# Autodesk Inventor assembly: Colmeia
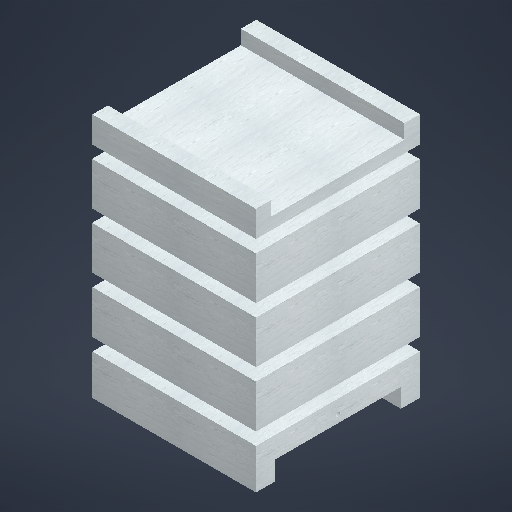
[picture p0: Inventor's stored thumbnail of the model, 512x512]
Saved by Autodesk Inventor 2027 (Build 310192000, 192)
## iProperties
Created: 2026-10-01
Part Number: Colmeia
Document SubType Name: Assembly
Designer: EspacoMaker
Author: EspacoMaker
## Documents named in this file (5)
- C:\Users\EspacoMaker\Documents\PeterIgnatious\BeeBox\3dFiles\Colmeia.iam
- C:\Users\EspacoMaker\Documents\PeterIgnatious\BeeBox\3dFiles\FundoColmeia.ipt
- C:\Users\EspacoMaker\Documents\PeterIgnatious\BeeBox\3dFiles\NinhoColmeia.ipt
- C:\Users\EspacoMaker\Documents\PeterIgnatious\BeeBox\3dFiles\Melgueira-Sobreninho.ipt
- C:\Users\EspacoMaker\Documents\PeterIgnatious\BeeBox\3dFiles\Tampa.ipt
## Components (5 placed, 4 different names)
1. FundoColmeia:1 — Coincidente:1, Alinhado:1, Alinhado:2
2. NinhoColmeia:1 — Coincidente:1, Alinhado:1, Alinhado:2, Coincidente:2, Alinhado:3, Alinhado:4
3. Melgueira-Sobreninho:1 — Coincidente:2, Alinhado:3, Alinhado:4, Coincidente:3, Alinhado:5, Alinhado:6
4. Melgueira-Sobreninho:2 — Coincidente:3, Alinhado:5, Alinhado:6, Coincidente:4, Alinhado:7, Alinhado:8
5. Tampa:1 — Coincidente:4, Alinhado:7, Alinhado:8
## Relationships (12: Flush 8, Mate 4)
- Coincidente:1 [Mate] (20 mm): FundoColmeia:1 ↔ NinhoColmeia:1
- Alinhado:1 [Flush]: FundoColmeia:1 ↔ NinhoColmeia:1
- Alinhado:2 [Flush]: FundoColmeia:1 ↔ NinhoColmeia:1
- Coincidente:2 [Mate] (20 mm): NinhoColmeia:1 ↔ Melgueira-Sobreninho:1
- Alinhado:3 [Flush]: NinhoColmeia:1 ↔ Melgueira-Sobreninho:1
- Alinhado:4 [Flush]: NinhoColmeia:1 ↔ Melgueira-Sobreninho:1
- Coincidente:3 [Mate] (20 mm): Melgueira-Sobreninho:1 ↔ Melgueira-Sobreninho:2
- Alinhado:5 [Flush]: Melgueira-Sobreninho:1 ↔ Melgueira-Sobreninho:2
- Alinhado:6 [Flush]: Melgueira-Sobreninho:1 ↔ Melgueira-Sobreninho:2
- Coincidente:4 [Mate] (20 mm): Melgueira-Sobreninho:2 ↔ Tampa:1
- Alinhado:7 [Flush]: Melgueira-Sobreninho:2 ↔ Tampa:1
- Alinhado:8 [Flush]: Melgueira-Sobreninho:2 ↔ Tampa:1
